# Autodesk Inventor assembly: arm
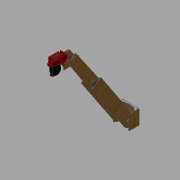
[picture p0: Inventor's stored thumbnail of the model, 180x180]
Saved by Autodesk Inventor 2013 (Build 170138000, 138)
## iProperties
Created: 2014-10-10
Part Number: arm
Document SubType Name: Assembly
Designer: Masta
Author: Masta
## Documents named in this file (7)
- D:\DrOctopus\3D model\arm\arm.iam
- D:\DrOctopus\3D model\arm\segment1.iam
- D:\DrOctopus\3D model\arm\segment2.iam
- D:\DrOctopus\3D model\arm\segment0.iam
- D:\DrOctopus\3D model\arm\segment3.iam
- D:\DrOctopus\3D model\arm\elektronika.ipt
- D:\DrOctopus\3D model\extruder\extruder.iam
## Components (6 placed, 6 different names)
1. segment1:1 [sub-assembly] — Insert:1, Insert:2, Angle:1, Angle:2, Mate:4, Flush:1, Flush:2
2. segment2:1 [sub-assembly] — Insert:1, Angle:1, Insert:3
3. segment0:1 [sub-assembly] — Insert:2, Angle:2, Flush:3, Mate:5, Mate:6
4. segment3:1 [sub-assembly] — Insert:3, Angle:4, Mate:7, Flush:4, Flush:5
5. elektronika:1 — Mate:4, Flush:1, Flush:2
6. extruder:1 [sub-assembly] — Mate:7, Flush:4, Flush:5
## Relationships (15: Flush 5, Mate 4, Insert 3, Angle 3)
- Insert:1: segment1:1 ↔ segment2:1
- Insert:2 (1 mm): segment1:1 ↔ segment0:1
- Angle:1 (30 deg): segment1:1 ↔ segment2:1
- Angle:2 (45 deg): segment1:1 ↔ segment0:1
- Insert:3: segment2:1 ↔ segment3:1
- Angle:4 (0 deg): segment3:1
- Mate:4: segment1:1 ↔ elektronika:1
- Flush:1 (10 mm): segment1:1 ↔ elektronika:1
- Flush:2 (100 mm): segment1:1 ↔ elektronika:1
- Flush:3: segment0:1
- Mate:5: segment0:1
- Mate:6: segment0:1
- Mate:7: segment3:1 ↔ extruder:1
- Flush:4: segment3:1 ↔ extruder:1
- Flush:5 (10 mm): segment3:1 ↔ extruder:1
